# Autodesk Inventor assembly: Light-Sheet Geometry
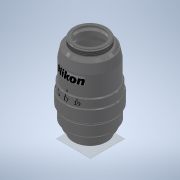
[picture p0: Inventor's stored thumbnail of the model, 180x180]
Saved by Autodesk Inventor 2022 (Build 260153000, 153)
## iProperties
Created: 2020-06-18
Part Number: Light-Sheet Geometry
Document SubType Name: Assembly
Designer: MicroscopyInnovation
Author: MicroscopyInnovation
## Documents named in this file (4)
- C:\Users\Spectral\Documents\GitHub\CAD\Manuscripts\Sapoznik-2020\Light-Sheet Geometry.iam
- C:\Users\Spectral\Documents\GitHub\CAD\Manuscripts\Sapoznik-2020\Nikon_DIC_N2_Objective.ipt
- C:\Users\Spectral\Documents\GitHub\CAD\Manuscripts\Sapoznik-2020\Glass.ipt
- C:\Users\Spectral\Documents\GitHub\CAD\Manuscripts\Sapoznik-2020\Light-Sheet.ipt
## Components (3 placed, 3 different names)
1. Nikon_DIC_N2_Objective:1 — Angle:1, Mate:1
2. Glass:1 — Angle:1, Mate:1, Angle:2, Angle:3, Mate:2
3. Light-Sheet:1 — Angle:2, Angle:3, Mate:2
## Relationships (5: Angle 3, Mate 2)
- Angle:1 (0 deg): Nikon_DIC_N2_Objective:1 ↔ Glass:1
- Mate:1 (0.1 mm): Nikon_DIC_N2_Objective:1 ↔ Glass:1
- Angle:2 (30 deg): Glass:1 ↔ Light-Sheet:1
- Angle:3 (0 deg): Glass:1 ↔ Light-Sheet:1
- Mate:2: Glass:1 ↔ Light-Sheet:1
